# Autodesk Inventor assembly: Gearboxes_001_assembly for 3
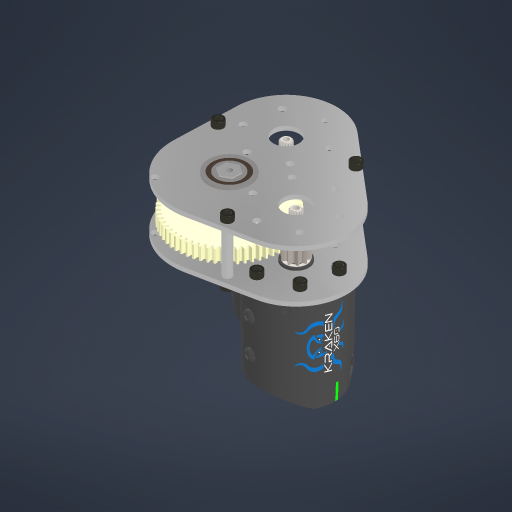
[picture p0: Inventor's stored thumbnail of the model, 512x512]
Saved by Autodesk Inventor 2024.4 (Build 284460000, 460)
## iProperties
Created: 2026-06-11
Part Number: Gearboxes_001_assembly for 3
Document SubType Name: Assembly
Designer: stanr
Author: stanr
## Documents named in this file (10)
- C:\Users\stanr\Documents\GitHub\2026-2027-DesignTraining\Stan\Gearboxes_001_assembly for 3.iam
- C:\Users\stanr\Documents\GitHub\2026-2027-DesignTraining\Stan\Gearboxes_3_thingy that holds motors and more.ipt
- C:\Users\stanr\Documents\GitHub\2026-2027-DesignTraining\COTS Library\Motors\COTS_WCP-0940_KrakenX60_New.ipt
- C:\Users\stanr\Documents\GitHub\2026-2027-DesignTraining\COTS Library\Motion\Bearings\COTS_WCP-0783_1.125ODHexBearing.ipt
- C:\Users\stanr\Documents\GitHub\2026-2027-DesignTraining\Stan\Gearboxes_003_standoff.ipt
- C:\Users\stanr\Documents\GitHub\2026-2027-DesignTraining\Stan\WCP-0720\WCP-0720.ipt
- C:\Users\stanr\Documents\GitHub\2026-2027-DesignTraining\Stan\WCP-0973\WCP-0973.ipt
- C:\Users\stanr\Documents\GitHub\2026-2027-DesignTraining\Stan\WCP-1008\WCP-1008\WCP-1008.ipt
- C:\Users\stanr\Documents\GitHub\2026-2027-DesignTraining\Stan\Gearboxes_002_Hexshaft my fav.ipt
- C:\Users\stanr\Documents\GitHub\2026-2027-DesignTraining\COTS Library\Fasteners\Bolts\Socket-Head\10-32\COTS_91251A342_1-2in Long_Black-Oxide Alloy Steel Socket Head.ipt
## Components (26 placed, 9 different names)
1. Gearboxes_3_thingy that holds motors and more:1 — Mate:1, Mate:2, Mate:3, Mate:4, Mate:5, Mate:6, Mate:7, Mate:9, Mate:10, Mate:11, Mate:12, Mate:13, Mate:15, Mate:16, Mate:44, Mate:45, Mate:46, Mate:47, Mate:48, Mate:50, Mate:51, Mate:52, Mate:53, Mate:55, Mate:56, Mate:57, Mate:58, Mate:60, Mate:61, Mate:62, Mate:63, Mate:64
2. COTS_WCP-0940_KrakenX60_New:1 — Mate:3, Mate:6, Mate:16, Mate:19, Mate:20
3. COTS_WCP-0940_KrakenX60_New:2 — Mate:4, Mate:5, Mate:15, Mate:17, Mate:18
4. COTS_WCP-0783_1.125ODHexBearing:1 — Mate:1, Mate:2, Mate:23, Mate:24, Mate:25
5. Gearboxes_003_standoff:1 — Mate:7, Mate:13
6. Gearboxes_003_standoff:2 — Mate:9, Mate:12
7. Gearboxes_003_standoff:4 — Mate:10, Mate:11, Mate:31
8. WCP-0720:1 — Mate:23, Mate:26, Mate:28
9. WCP-0973:1 — Mate:27, Mate:28
10. WCP-1008:1 — Mate:17, Mate:18
11. WCP-1008:2 — Mate:19, Mate:20
12. Gearboxes_3_thingy that holds motors and more:2 — Mate:31, Mate:32, Mate:33, Mate:34, Mate:35, Mate:36, Mate:37, Mate:41, Mate:42
13. Gearboxes_002_Hexshaft my fav:2 — Mate:24, Mate:25, Mate:26, Mate:27
14. COTS_WCP-0783_1.125ODHexBearing:2 — Mate:32, Mate:33
15. COTS_91251A342_1-2in Long_Black-Oxide Alloy Steel Socket Head:1 — Mate:53, Mate:62
16. COTS_91251A342_1-2in Long_Black-Oxide Alloy Steel Socket Head:2 — Mate:52, Mate:60
17. COTS_91251A342_1-2in Long_Black-Oxide Alloy Steel Socket Head:3 — Mate:51, Mate:61
18. COTS_91251A342_1-2in Long_Black-Oxide Alloy Steel Socket Head:5 — Mate:34, Mate:35
19. COTS_91251A342_1-2in Long_Black-Oxide Alloy Steel Socket Head:6 — Mate:36, Mate:37
20. COTS_91251A342_1-2in Long_Black-Oxide Alloy Steel Socket Head:8 — Mate:41, Mate:42
21. COTS_91251A342_1-2in Long_Black-Oxide Alloy Steel Socket Head:9 — Mate:44, Mate:48
22. COTS_91251A342_1-2in Long_Black-Oxide Alloy Steel Socket Head:11 — Mate:46, Mate:47
23. COTS_91251A342_1-2in Long_Black-Oxide Alloy Steel Socket Head:12 — Mate:45, Mate:50
24. COTS_91251A342_1-2in Long_Black-Oxide Alloy Steel Socket Head:13 — Mate:56, Mate:57
25. COTS_91251A342_1-2in Long_Black-Oxide Alloy Steel Socket Head:15 — Mate:55, Mate:58
26. COTS_91251A342_1-2in Long_Black-Oxide Alloy Steel Socket Head:16 — Mate:63, Mate:64
## Relationships (51: Mate 51)
- Mate:1: Gearboxes_3_thingy that holds motors and more:1 ↔ COTS_WCP-0783_1.125ODHexBearing:1
- Mate:2: Gearboxes_3_thingy that holds motors and more:1 ↔ COTS_WCP-0783_1.125ODHexBearing:1
- Mate:3: Gearboxes_3_thingy that holds motors and more:1 ↔ COTS_WCP-0940_KrakenX60_New:1
- Mate:4: Gearboxes_3_thingy that holds motors and more:1 ↔ COTS_WCP-0940_KrakenX60_New:2
- Mate:5: Gearboxes_3_thingy that holds motors and more:1 ↔ COTS_WCP-0940_KrakenX60_New:2
- Mate:6: Gearboxes_3_thingy that holds motors and more:1 ↔ COTS_WCP-0940_KrakenX60_New:1
- Mate:7: Gearboxes_3_thingy that holds motors and more:1 ↔ Gearboxes_003_standoff:1
- Mate:9: Gearboxes_3_thingy that holds motors and more:1 ↔ Gearboxes_003_standoff:2
- Mate:10: Gearboxes_3_thingy that holds motors and more:1 ↔ Gearboxes_003_standoff:4
- Mate:11: Gearboxes_3_thingy that holds motors and more:1 ↔ Gearboxes_003_standoff:4
- Mate:12: Gearboxes_3_thingy that holds motors and more:1 ↔ Gearboxes_003_standoff:2
- Mate:13: Gearboxes_3_thingy that holds motors and more:1 ↔ Gearboxes_003_standoff:1
- Mate:15: Gearboxes_3_thingy that holds motors and more:1 ↔ COTS_WCP-0940_KrakenX60_New:2
- Mate:16: Gearboxes_3_thingy that holds motors and more:1 ↔ COTS_WCP-0940_KrakenX60_New:1
- Mate:17: COTS_WCP-0940_KrakenX60_New:2 ↔ WCP-1008:1
- Mate:18: COTS_WCP-0940_KrakenX60_New:2 ↔ WCP-1008:1
- Mate:19: COTS_WCP-0940_KrakenX60_New:1 ↔ WCP-1008:2
- Mate:20: COTS_WCP-0940_KrakenX60_New:1 ↔ WCP-1008:2
- Mate:23: COTS_WCP-0783_1.125ODHexBearing:1 ↔ WCP-0720:1
- Mate:24: COTS_WCP-0783_1.125ODHexBearing:1 ↔ Gearboxes_002_Hexshaft my fav:2
- Mate:25: COTS_WCP-0783_1.125ODHexBearing:1 ↔ Gearboxes_002_Hexshaft my fav:2
- Mate:26: WCP-0720:1 ↔ Gearboxes_002_Hexshaft my fav:2
- Mate:27: WCP-0973:1 ↔ Gearboxes_002_Hexshaft my fav:2
- Mate:28: WCP-0720:1 ↔ WCP-0973:1
- Mate:31: Gearboxes_003_standoff:4 ↔ Gearboxes_3_thingy that holds motors and more:2
- Mate:32: Gearboxes_3_thingy that holds motors and more:2 ↔ COTS_WCP-0783_1.125ODHexBearing:2
- Mate:33: Gearboxes_3_thingy that holds motors and more:2 ↔ COTS_WCP-0783_1.125ODHexBearing:2
- Mate:34: Gearboxes_3_thingy that holds motors and more:2 ↔ COTS_91251A342_1-2in Long_Black-Oxide Alloy Steel Socket Head:5
- Mate:35: Gearboxes_3_thingy that holds motors and more:2 ↔ COTS_91251A342_1-2in Long_Black-Oxide Alloy Steel Socket Head:5
- Mate:36: Gearboxes_3_thingy that holds motors and more:2 ↔ COTS_91251A342_1-2in Long_Black-Oxide Alloy Steel Socket Head:6
- Mate:37: Gearboxes_3_thingy that holds motors and more:2 ↔ COTS_91251A342_1-2in Long_Black-Oxide Alloy Steel Socket Head:6
- Mate:41: Gearboxes_3_thingy that holds motors and more:2 ↔ COTS_91251A342_1-2in Long_Black-Oxide Alloy Steel Socket Head:8
- Mate:42: Gearboxes_3_thingy that holds motors and more:2 ↔ COTS_91251A342_1-2in Long_Black-Oxide Alloy Steel Socket Head:8
- Mate:44: Gearboxes_3_thingy that holds motors and more:1 ↔ COTS_91251A342_1-2in Long_Black-Oxide Alloy Steel Socket Head:9
- Mate:45: Gearboxes_3_thingy that holds motors and more:1 ↔ COTS_91251A342_1-2in Long_Black-Oxide Alloy Steel Socket Head:12
- Mate:46: Gearboxes_3_thingy that holds motors and more:1 ↔ COTS_91251A342_1-2in Long_Black-Oxide Alloy Steel Socket Head:11
- Mate:47: Gearboxes_3_thingy that holds motors and more:1 ↔ COTS_91251A342_1-2in Long_Black-Oxide Alloy Steel Socket Head:11
- Mate:48: Gearboxes_3_thingy that holds motors and more:1 ↔ COTS_91251A342_1-2in Long_Black-Oxide Alloy Steel Socket Head:9
- Mate:50: Gearboxes_3_thingy that holds motors and more:1 ↔ COTS_91251A342_1-2in Long_Black-Oxide Alloy Steel Socket Head:12
- Mate:51: Gearboxes_3_thingy that holds motors and more:1 ↔ COTS_91251A342_1-2in Long_Black-Oxide Alloy Steel Socket Head:3
- Mate:52: Gearboxes_3_thingy that holds motors and more:1 ↔ COTS_91251A342_1-2in Long_Black-Oxide Alloy Steel Socket Head:2
- Mate:53: Gearboxes_3_thingy that holds motors and more:1 ↔ COTS_91251A342_1-2in Long_Black-Oxide Alloy Steel Socket Head:1
- Mate:55: Gearboxes_3_thingy that holds motors and more:1 ↔ COTS_91251A342_1-2in Long_Black-Oxide Alloy Steel Socket Head:15
- Mate:56: Gearboxes_3_thingy that holds motors and more:1 ↔ COTS_91251A342_1-2in Long_Black-Oxide Alloy Steel Socket Head:13
- Mate:57: Gearboxes_3_thingy that holds motors and more:1 ↔ COTS_91251A342_1-2in Long_Black-Oxide Alloy Steel Socket Head:13
- Mate:58: Gearboxes_3_thingy that holds motors and more:1 ↔ COTS_91251A342_1-2in Long_Black-Oxide Alloy Steel Socket Head:15
- Mate:60: Gearboxes_3_thingy that holds motors and more:1 ↔ COTS_91251A342_1-2in Long_Black-Oxide Alloy Steel Socket Head:2
- Mate:61: Gearboxes_3_thingy that holds motors and more:1 ↔ COTS_91251A342_1-2in Long_Black-Oxide Alloy Steel Socket Head:3
- Mate:62: Gearboxes_3_thingy that holds motors and more:1 ↔ COTS_91251A342_1-2in Long_Black-Oxide Alloy Steel Socket Head:1
- Mate:63: Gearboxes_3_thingy that holds motors and more:1 ↔ COTS_91251A342_1-2in Long_Black-Oxide Alloy Steel Socket Head:16
- Mate:64: Gearboxes_3_thingy that holds motors and more:1 ↔ COTS_91251A342_1-2in Long_Black-Oxide Alloy Steel Socket Head:16
